# Autodesk Inventor assembly: CARCASA_ESTRUCTURA_Y_CHAPAS
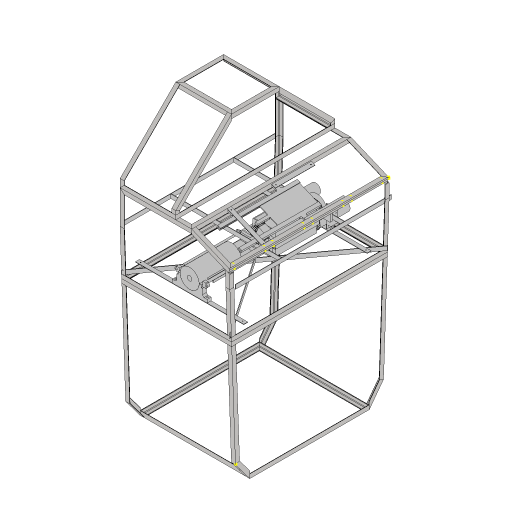
[picture p0: Inventor's stored thumbnail of the model, 512x512]
Saved by Autodesk Inventor 2024 (Build 280153000, 153)
## iProperties
Created: 2024-05-18
Part Number: CARCASA_ESTRUCTURA_Y_CHAPAS
Material: Generic
Document SubType Name: Assembly
Designer: Niler
Author: Niler
## Documents named in this file (7)
- C:\Users\Jhuliams\Documents\GitHub\RECICLADOR_MODELO_3D\VERSION_3_COMPLETA\CARCASA_ESTRUCTURA_Y_CHAPAS.iam
- C:\Users\Jhuliams\Documents\GitHub\RECICLADOR_MODELO_3D\VERSION_3_COMPLETA\ESTRUCTURA\ESTRUCTURA_COMPLETA.iam
- C:\Users\Jhuliams\Documents\GitHub\RECICLADOR_MODELO_3D\MECANISMO DE COMPACTADO\ENSAMBLE MECANISMO DE INGRESO.iam
- C:\Users\Jhuliams\Documents\GitHub\RECICLADOR_MODELO_3D\MECANISMO DE COMPACTADO\MECANISMO DE COMPACTADO.iam
- C:\Users\Jhuliams\Documents\GitHub\RECICLADOR_MODELO_3D\MECANISMO DE COMPACTADO\PLETINA DE INERCIA.ipt
- C:\Users\Jhuliams\Documents\GitHub\RECICLADOR_MODELO_3D\MECANISMO DE COMPACTADO\SEPARACION LATA-BOTELLA Y PAPEL.iam
- C:\Users\Jhuliams\Documents\GitHub\RECICLADOR_MODELO_3D\MECANISMO DE COMPACTADO\SOPORTE INERCIAL DE LA CAJA SEPARADORA.ipt
## Components (6 placed, 6 different names)
1. ESTRUCTURA_COMPLETA:1 [sub-assembly] — Mate:1, Mate:2, Mate:4, Mate:7, Mate:8, Mate:9, Mate:10, Mate:11, Mate:13
2. ENSAMBLE MECANISMO DE INGRESO:1 [sub-assembly] — Mate:1, Mate:2, Mate:5
3. MECANISMO DE COMPACTADO:1 [sub-assembly] — Mate:4, Mate:5, Mate:6, Mate:8
4. PLETINA DE INERCIA:1 — Mate:6, Mate:7
5. SEPARACION LATA-BOTELLA Y PAPEL:1 [sub-assembly] — Mate:9, Mate:10, Mate:11, Mate:12, Flush:1
6. SOPORTE INERCIAL DE LA CAJA SEPARADORA:1 — Mate:12, Mate:13, Flush:1
## Relationships (13: Mate 12, Flush 1)
- Mate:1: ESTRUCTURA_COMPLETA:1 ↔ ENSAMBLE MECANISMO DE INGRESO:1
- Mate:2 (224.6 mm): ESTRUCTURA_COMPLETA:1 ↔ ENSAMBLE MECANISMO DE INGRESO:1
- Mate:4: ESTRUCTURA_COMPLETA:1 ↔ MECANISMO DE COMPACTADO:1
- Mate:5: ENSAMBLE MECANISMO DE INGRESO:1 ↔ MECANISMO DE COMPACTADO:1
- Mate:6: MECANISMO DE COMPACTADO:1 ↔ PLETINA DE INERCIA:1
- Mate:7: ESTRUCTURA_COMPLETA:1 ↔ PLETINA DE INERCIA:1
- Mate:8 (50 mm): ESTRUCTURA_COMPLETA:1 ↔ MECANISMO DE COMPACTADO:1
- Mate:9 (220 mm): ESTRUCTURA_COMPLETA:1 ↔ SEPARACION LATA-BOTELLA Y PAPEL:1
- Mate:10 (100 mm): ESTRUCTURA_COMPLETA:1 ↔ SEPARACION LATA-BOTELLA Y PAPEL:1
- Mate:11 (349 mm): ESTRUCTURA_COMPLETA:1 ↔ SEPARACION LATA-BOTELLA Y PAPEL:1
- Mate:12: SEPARACION LATA-BOTELLA Y PAPEL:1 ↔ SOPORTE INERCIAL DE LA CAJA SEPARADORA:1
- Mate:13: ESTRUCTURA_COMPLETA:1 ↔ SOPORTE INERCIAL DE LA CAJA SEPARADORA:1
- Flush:1 (9.25 mm): SEPARACION LATA-BOTELLA Y PAPEL:1 ↔ SOPORTE INERCIAL DE LA CAJA SEPARADORA:1
